# Autodesk Inventor assembly: High Strength Chain Generator
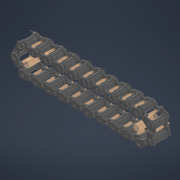
[picture p0: Inventor's stored thumbnail of the model, 180x180]
Saved by Autodesk Inventor 2021 (Build 250183000, 183)
## iProperties
RuleStatus: InUse
Created: 2020-07-07
Part Number: High Strength Chain Generator
Document SubType Name: Assembly
Designer: yuany
AfterDocOpen0: Open Form
Author: yuany
## Documents named in this file (9)
- C:\Users\Robotics\Desktop\CAD\Library 1.2\Motion\Chain + Tank Tread\Parametric\High Strength Chain Generator.iam
- C:\Users\Robotics\Desktop\CAD\Library 1.2\Motion\Chain + Tank Tread\Parametric\Workpoint Pattern.ipt
- C:\Users\Robotics\Desktop\CAD\Library 1.1\Motion\Chain + Tank Tread\High Strength Chain Link.ipt
- C:\Users\Robotics\Desktop\CAD\Library 1.1\Motion\Chain + Tank Tread\Tank Tread Traction Link.ipt
- C:\Users\Robotics\Desktop\CAD\Library 1.1\Motion\Chain + Tank Tread\Tread Link.ipt
- C:\Users\Robotics\Desktop\CAD\Library 1.1\Motion\Chain + Tank Tread\Chain Attachment Link.ipt
- C:\Users\Robotics\Desktop\CAD\Library 1.2\Motion\Chain + Tank Tread\Short Flap.ipt
- C:\Users\Robotics\Desktop\CAD\Library 1.2\Motion\Chain + Tank Tread\Medium Flap.ipt
- C:\Users\Robotics\Desktop\CAD\Library 1.2\Motion\Chain + Tank Tread\Tall Flap.ipt
## Components (162 placed, 8 different names)
1. Workpoint Pattern:3 — Mate:1, Mate:2, Mate:3
2. High Strength Chain Link:1 — Mate:1, Mate:2, Mate:3, Flush:1, Mate:4, Angle:1
3. High Strength Chain Link:2
4. High Strength Chain Link:3
5. High Strength Chain Link:4
6. High Strength Chain Link:5
7. High Strength Chain Link:6
8. High Strength Chain Link:7
9. High Strength Chain Link:8
10. High Strength Chain Link:9
11. High Strength Chain Link:10
12. High Strength Chain Link:11
13. High Strength Chain Link:12
14. High Strength Chain Link:13
15. High Strength Chain Link:14
16. High Strength Chain Link:15
17. High Strength Chain Link:16
18. High Strength Chain Link:17
19. High Strength Chain Link:18
20. High Strength Chain Link:19
21. High Strength Chain Link:20
22. High Strength Chain Link:21
23. High Strength Chain Link:22
24. High Strength Chain Link:23
25. Tank Tread Traction Link:1 — Flush:1, Mate:4, Angle:1, Flush:2, Mate:5, Angle:2
26. Tank Tread Traction Link:2
27. Tank Tread Traction Link:3
28. Tank Tread Traction Link:4
29. Tank Tread Traction Link:5
30. Tank Tread Traction Link:6
31. Tank Tread Traction Link:7
32. Tank Tread Traction Link:8
33. Tank Tread Traction Link:9
34. Tank Tread Traction Link:10
35. Tank Tread Traction Link:11
36. Tank Tread Traction Link:12
37. Tank Tread Traction Link:13
38. Tank Tread Traction Link:14
39. Tank Tread Traction Link:15
40. Tank Tread Traction Link:16
41. Tank Tread Traction Link:17
42. Tank Tread Traction Link:18
43. Tank Tread Traction Link:19
44. Tank Tread Traction Link:20
45. Tank Tread Traction Link:21
46. Tank Tread Traction Link:22
47. Tank Tread Traction Link:23
48. Tread Link:1 — Flush:2, Mate:5, Angle:2, Flush:3, Mate:6, Angle:3
49. Tread Link:2
50. Tread Link:3
51. Tread Link:4
52. Tread Link:5
53. Tread Link:6
54. Tread Link:7
55. Tread Link:8
56. Tread Link:9
57. Tread Link:10
58. Tread Link:11
59. Tread Link:12
60. Tread Link:13
61. Tread Link:14
62. Tread Link:15
63. Tread Link:16
64. Tread Link:17
65. Tread Link:18
66. Tread Link:19
67. Tread Link:20
68. Tread Link:21
69. Tread Link:22
70. Tread Link:23
71. Chain Attachment Link:1 — Flush:3, Mate:6, Angle:3
72. Chain Attachment Link:2
73. Chain Attachment Link:3
74. Chain Attachment Link:4
75. Chain Attachment Link:5
76. Chain Attachment Link:6
77. Chain Attachment Link:7
78. Chain Attachment Link:8
79. Chain Attachment Link:9
80. Chain Attachment Link:10
81. Chain Attachment Link:11
82. Chain Attachment Link:12
83. Chain Attachment Link:13
84. Chain Attachment Link:14
85. Chain Attachment Link:15
86. Chain Attachment Link:16
87. Chain Attachment Link:17
88. Chain Attachment Link:18
89. Chain Attachment Link:19
90. Chain Attachment Link:20
91. Chain Attachment Link:21
92. Chain Attachment Link:22
93. Chain Attachment Link:23
94. Short Flap:1 [sub-assembly]
95. Short Flap:2 [sub-assembly]
96. Short Flap:3 [sub-assembly]
97. Short Flap:4 [sub-assembly]
98. Short Flap:5 [sub-assembly]
99. Short Flap:6 [sub-assembly]
100. Short Flap:7 [sub-assembly]
101. Short Flap:8 [sub-assembly]
102. Short Flap:9 [sub-assembly]
103. Short Flap:10 [sub-assembly]
104. Short Flap:11 [sub-assembly]
105. Short Flap:12 [sub-assembly]
106. Short Flap:13 [sub-assembly]
107. Short Flap:14 [sub-assembly]
108. Short Flap:15 [sub-assembly]
109. Short Flap:16 [sub-assembly]
110. Short Flap:17 [sub-assembly]
111. Short Flap:18 [sub-assembly]
112. Short Flap:19 [sub-assembly]
113. Short Flap:20 [sub-assembly]
114. Short Flap:21 [sub-assembly]
115. Short Flap:22 [sub-assembly]
116. Short Flap:23 [sub-assembly]
117. Medium Flap:1 [sub-assembly]
118. Medium Flap:2 [sub-assembly]
119. Medium Flap:3 [sub-assembly]
120. Medium Flap:4 [sub-assembly]
121. Medium Flap:5 [sub-assembly]
122. Medium Flap:6 [sub-assembly]
123. Medium Flap:7 [sub-assembly]
124. Medium Flap:8 [sub-assembly]
125. Medium Flap:9 [sub-assembly]
126. Medium Flap:10 [sub-assembly]
127. Medium Flap:11 [sub-assembly]
128. Medium Flap:12 [sub-assembly]
129. Medium Flap:13 [sub-assembly]
130. Medium Flap:14 [sub-assembly]
131. Medium Flap:15 [sub-assembly]
132. Medium Flap:16 [sub-assembly]
133. Medium Flap:17 [sub-assembly]
134. Medium Flap:18 [sub-assembly]
135. Medium Flap:19 [sub-assembly]
136. Medium Flap:20 [sub-assembly]
137. Medium Flap:21 [sub-assembly]
138. Medium Flap:22 [sub-assembly]
139. Medium Flap:23 [sub-assembly]
140. Tall Flap:1 [sub-assembly]
141. Tall Flap:2 [sub-assembly]
142. Tall Flap:3 [sub-assembly]
143. Tall Flap:4 [sub-assembly]
144. Tall Flap:5 [sub-assembly]
145. Tall Flap:6 [sub-assembly]
146. Tall Flap:7 [sub-assembly]
147. Tall Flap:8 [sub-assembly]
148. Tall Flap:9 [sub-assembly]
149. Tall Flap:10 [sub-assembly]
150. Tall Flap:11 [sub-assembly]
151. Tall Flap:12 [sub-assembly]
152. Tall Flap:13 [sub-assembly]
153. Tall Flap:14 [sub-assembly]
154. Tall Flap:15 [sub-assembly]
155. Tall Flap:16 [sub-assembly]
156. Tall Flap:17 [sub-assembly]
157. Tall Flap:18 [sub-assembly]
158. Tall Flap:19 [sub-assembly]
159. Tall Flap:20 [sub-assembly]
160. Tall Flap:21 [sub-assembly]
161. Tall Flap:22 [sub-assembly]
162. Tall Flap:23 [sub-assembly]
## Component patterns: Chain (23 elements), Traction (23 elements), Tread (23 elements), Chain Attachment (23 elements), Short Flaps (23 elements), Medium Flaps (23 elements), Tall Flaps (23 elements)
## Relationships (12: Mate 6, Flush 3, Angle 3)
- Mate:1: Workpoint Pattern:3 ↔ High Strength Chain Link:1
- Mate:2 (11.938 mm): Workpoint Pattern:3 ↔ High Strength Chain Link:1
- Mate:3: Workpoint Pattern:3 ↔ High Strength Chain Link:1
- Flush:1: High Strength Chain Link:1 ↔ Tank Tread Traction Link:1
- Mate:4: High Strength Chain Link:1 ↔ Tank Tread Traction Link:1
- Angle:1 (180 deg): High Strength Chain Link:1 ↔ Tank Tread Traction Link:1
- Flush:2: Tank Tread Traction Link:1 ↔ Tread Link:1
- Mate:5: Tank Tread Traction Link:1 ↔ Tread Link:1
- Angle:2 (0 deg): Tank Tread Traction Link:1 ↔ Tread Link:1
- Flush:3: Tread Link:1 ↔ Chain Attachment Link:1
- Mate:6: Tread Link:1 ↔ Chain Attachment Link:1
- Angle:3 (0 deg): Tread Link:1 ↔ Chain Attachment Link:1
## Named parameters: Center_Distance = 88.9 mm, Sprocket1 = 19.558 mm, Sprocket2 = 19.558 mm, CenterDistance = 88.9 mm, d5_1 = 88.9 mm, d6_1 = 88.9 mm, d7_1 = 30.72163 mm, d8_1 = 30.72163 mm
